# Autodesk Inventor assembly: Roller_Bracket
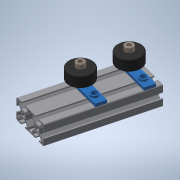
[picture p0: Inventor's stored thumbnail of the model, 180x180]
Saved by Autodesk Inventor 2021 (Build 250183000, 183)
## iProperties
Created: 2021-02-01
Part Number: Roller_Bracket
Document SubType Name: Assembly
Designer: Jorian Brusind
Mass: 44.0669 g
Surface Area: 169.812 cm^2
Volume: 42.4218 cm^3
Density: 1.03878 g/cm^3
Author: Jorian Brusind
## Documents named in this file (5)
- C:\Users\Jorian Brusind\Documents\GitHub\PersonalProjects\HyperRail\Inventor Files\Roller_Bracket.iam
- C:\Users\Jorian Brusind\Documents\GitHub\PersonalProjects\HyperRail\Inventor Files\11mm_BearingWheel.ipt
- C:\Users\Jorian Brusind\Documents\GitHub\PersonalProjects\Inventor Projects\Useful models\Metric bolt\Bolt M5 20mm.ipt
- C:\Users\Jorian Brusind\Documents\GitHub\PersonalProjects\Inventor Projects\Useful models\8020_Sets\IPT_20_Series\IPT_20_Series\20-2040_150mm.ipt
- C:\Users\Jorian Brusind\Documents\GitHub\PersonalProjects\HyperRail\Inventor Files\4mm_Roller_Spacer.ipt
## Components (7 placed, 4 different names)
1. 11mm_BearingWheel:1 — Mate:2, Mate:4, Mate:19
2. 11mm_BearingWheel:2 — Mate:6, Mate:8, Mate:18, Mate:20
3. Bolt M5 20mm:1 — Mate:6, Mate:8, Mate:15
4. Bolt M5 20mm:2 — Mate:2, Mate:4, Mate:13
5. 20-2040_150mm:1 — Mate:12, Angle:1, Flush:1, Mate:14, Flush:2, Mate:20
6. 4mm_Roller_Spacer:1 — Mate:14, Flush:2, Mate:15, Mate:17, Mate:18
7. 4mm_Roller_Spacer:2 — Mate:12, Mate:13, Angle:1, Flush:1, Mate:17, Mate:19
## Relationships (15: Mate 12, Flush 2, Angle 1)
- Mate:2: 11mm_BearingWheel:1 ↔ Bolt M5 20mm:2
- Mate:4: 11mm_BearingWheel:1 ↔ Bolt M5 20mm:2
- Mate:6: 11mm_BearingWheel:2 ↔ Bolt M5 20mm:1
- Mate:8: 11mm_BearingWheel:2 ↔ Bolt M5 20mm:1
- Mate:12: 20-2040_150mm:1 ↔ 4mm_Roller_Spacer:2
- Mate:13: Bolt M5 20mm:2 ↔ 4mm_Roller_Spacer:2
- Angle:1 (0 deg): 20-2040_150mm:1 ↔ 4mm_Roller_Spacer:2
- Flush:1: 20-2040_150mm:1 ↔ 4mm_Roller_Spacer:2
- Mate:14: 20-2040_150mm:1 ↔ 4mm_Roller_Spacer:1
- Flush:2: 20-2040_150mm:1 ↔ 4mm_Roller_Spacer:1
- Mate:15: Bolt M5 20mm:1 ↔ 4mm_Roller_Spacer:1
- Mate:17 (31 mm): 4mm_Roller_Spacer:1 ↔ 4mm_Roller_Spacer:2
- Mate:18: 11mm_BearingWheel:2 ↔ 4mm_Roller_Spacer:1
- Mate:19: 11mm_BearingWheel:1 ↔ 4mm_Roller_Spacer:2
- Mate:20 (-11 mm): 11mm_BearingWheel:2 ↔ 20-2040_150mm:1
